# Autodesk Inventor assembly: 3D Print me
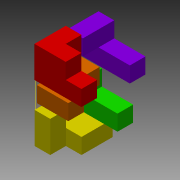
[picture p0: Inventor's stored thumbnail of the model, 180x180]
Saved by Autodesk Inventor 2014 (Build 180170000, 170)
## iProperties
Created: 2014-07-25
Part Number: 3D Print me
Document SubType Name: Assembly
Designer: quinn
Author: quinn
## Documents named in this file (6)
- C:\Quinn\Grabcad\Puzzle Cube\3D Print me.iam
- C:\Quinn\Grabcad\Puzzle Cube\Part1-01.ipt
- C:\Quinn\Grabcad\Puzzle Cube\Part2.ipt
- C:\Quinn\Grabcad\Puzzle Cube\Part3.ipt
- C:\Quinn\Grabcad\Puzzle Cube\Part4.ipt
- C:\Quinn\Grabcad\Puzzle Cube\Part5.ipt
## Components (5 placed, 5 different names)
1. Part1-01:1 — Mate:1, Mate:2, Mate:3
2. Part2:1 — Mate:4, Mate:9, Mate:10
3. Part4:1 — Mate:7
4. Part5:1 — Mate:6
5. Part3:1 — Mate:8, Mate:9, Mate:10
## Relationships (9: Mate 9)
- Mate:1: Part1-01:1
- Mate:2: Part1-01:1
- Mate:3: Part1-01:1
- Mate:4: Part2:1
- Mate:6: Part5:1
- Mate:7: Part4:1
- Mate:8: Part3:1
- Mate:9: Part2:1 ↔ Part3:1
- Mate:10: Part2:1 ↔ Part3:1
